# Autodesk Inventor assembly: VNA-Port1-Kabelfixierung
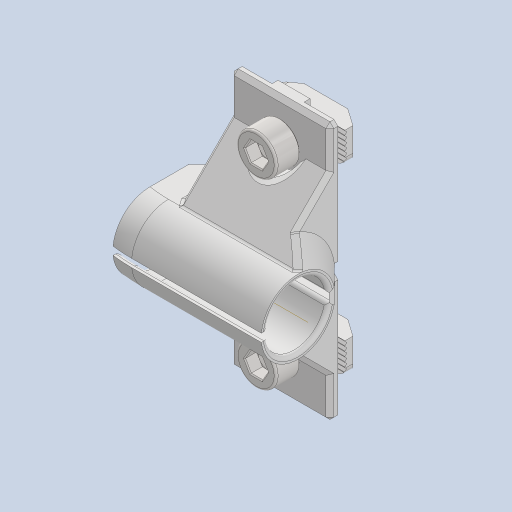
[picture p0: Inventor's stored thumbnail of the model, 512x512]
Saved by Autodesk Inventor 2023.2 (Build 272271000, 271)
## iProperties
Created: 2024-07-03
Part Number: VNA-Port1-Kabelfixierung
Document SubType Name: Assembly
Designer: Nils Bade
Author: Nils Bade
## Documents named in this file (4)
- C:\Users\nilsb\Documents\Inventor\Projektarbeit-Bade\RatRig_modified\VNA-Port1-Kabelfixierung.iam
- C:\Users\nilsb\Documents\Inventor\Projektarbeit-Bade\RatRig_modified\VNA-Port1-Kabelfixierung.ipt
- C:\Users\nilsb\Documents\Inventor\Projektarbeit-Bade\Schrauben\Cap Head Screw M6x12 v2.ipt
- C:\Users\nilsb\Documents\Inventor\Projektarbeit-Bade\RatRig_modified\T-NUT - DropIn 4040 SERIES - M6.ipt
## Components (5 placed, 3 different names)
1. VNA-Port1-Kabelfixierung:1 — Passend:1, Passend:2, Passend:3, Passend:4, Passend:5, Winkel:1, Winkel:2, Passend:8, Passend:9
2. Cap Head Screw M6x12 v2:1 — Passend:2, Passend:4, Passend:6
3. Cap Head Screw M6x12 v2:2 — Passend:3, Passend:5, Passend:7
4. T-NUT - DROP IN TYPE FOR 40 SERIES - M6:1 — Passend:6, Winkel:1, Passend:8
5. T-NUT - DROP IN TYPE FOR 40 SERIES - M6:2 — Passend:7, Winkel:2, Passend:9
## Relationships (11: Mate 9, Angle 2)
- Passend:1 [Mate]: VNA-Port1-Kabelfixierung:1
- Passend:2 [Mate]: VNA-Port1-Kabelfixierung:1 ↔ Cap Head Screw M6x12 v2:1
- Passend:3 [Mate]: VNA-Port1-Kabelfixierung:1 ↔ Cap Head Screw M6x12 v2:2
- Passend:4 [Mate]: VNA-Port1-Kabelfixierung:1 ↔ Cap Head Screw M6x12 v2:1
- Passend:5 [Mate]: VNA-Port1-Kabelfixierung:1 ↔ Cap Head Screw M6x12 v2:2
- Passend:6 [Mate]: Cap Head Screw M6x12 v2:1 ↔ T-NUT - DROP IN TYPE FOR 40 SERIES - M6:1
- Passend:7 [Mate]: Cap Head Screw M6x12 v2:2 ↔ T-NUT - DROP IN TYPE FOR 40 SERIES - M6:2
- Winkel:1 [Angle] (0 deg): VNA-Port1-Kabelfixierung:1 ↔ T-NUT - DROP IN TYPE FOR 40 SERIES - M6:1
- Winkel:2 [Angle] (0 deg): VNA-Port1-Kabelfixierung:1 ↔ T-NUT - DROP IN TYPE FOR 40 SERIES - M6:2
- Passend:8 [Mate] (4.5 mm): VNA-Port1-Kabelfixierung:1 ↔ T-NUT - DROP IN TYPE FOR 40 SERIES - M6:1
- Passend:9 [Mate] (4.5 mm): VNA-Port1-Kabelfixierung:1 ↔ T-NUT - DROP IN TYPE FOR 40 SERIES - M6:2
